# Autodesk Inventor assembly: Ensamble herramienta
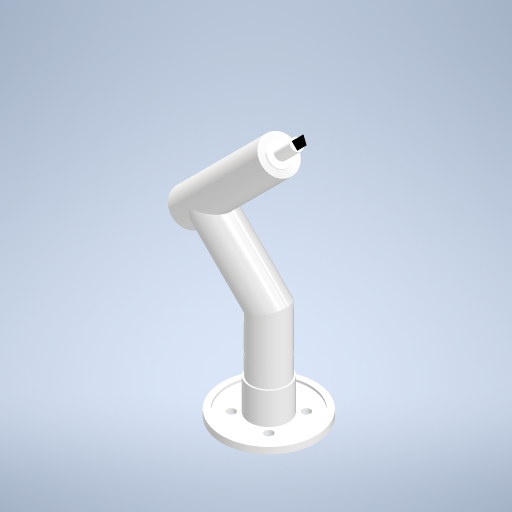
[picture p0: Inventor's stored thumbnail of the model, 512x512]
Saved by Autodesk Inventor 2024 (Build 280153000, 153)
## iProperties
Created: 2023-02-27
Part Number: Ensamble herramienta
Document SubType Name: Assembly
Designer: Braya
Mass: 168.022 g
Surface Area: 993.637 cm^2
Volume: 153.901 cm^3
Density: 1.09176 g/cm^3
Author: Braya
## Documents named in this file (6)
- C:\Users\profe\Downloads\Modelo-20230827T203604Z-001\Modelo\Ensamble herramienta.iam
- C:\Users\profe\Downloads\Modelo-20230827T203604Z-001\Modelo\Acople con rosca.ipt
- C:\Users\profe\Downloads\Modelo-20230827T203604Z-001\Modelo\Flanche.ipt
- C:\Users\profe\Downloads\Modelo-20230827T203604Z-001\Modelo\Semicodo.ipt
- C:\Users\profe\Downloads\Modelo-20230827T203604Z-001\Modelo\T.ipt
- C:\Users\profe\Downloads\Modelo-20230827T203604Z-001\Modelo\Marcador.ipt
## Components (5 placed, 5 different names)
1. Acople con rosca:1 — Insertar:1
2. Semicodo:1 — Coincidencia:3
3. T:1 — Coincidencia:3, Insertar:2
4. Flanche:1 — Insertar:1
5. Marcador:1 — Insertar:2
## Relationships (3: Insert 2, Mate 1)
- Coincidencia:3 [Mate]: Semicodo:1 ↔ T:1
- Insertar:1: Acople con rosca:1 ↔ Flanche:1
- Insertar:2: T:1 ↔ Marcador:1
